# Autodesk Inventor assembly: Assembly
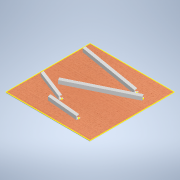
[picture p0: Inventor's stored thumbnail of the model, 180x180]
Saved by Autodesk Inventor 2020 (Build 240168000, 168)
## iProperties
Created: 2020-02-20
Part Number: Assembly
Document SubType Name: Assembly
Designer: brand
Author: brand
## Documents named in this file (3)
- C:\Users\brand\Documents\Longhorn 3D Printing\Week1\Inventor\Assembly.iam
- C:\Users\brand\Documents\Longhorn 3D Printing\Week1\Inventor\Base.ipt
- C:\Users\brand\Documents\Longhorn 3D Printing\Week1\Inventor\StraightTrackv2.ipt
## Components (7 placed, 2 different names)
1. Base:1 — Mate:1, Mate:2, Mate:3, Mate:4, Mate:5, Mate:6
2. StraightTrackv2:1 — Mate:1, Rigid:1
3. StraightTrackv2:2 — Mate:2, Rigid:1
4. StraightTrackv2:3 — Mate:5
5. StraightTrackv2:4 — Mate:3, Mate:7, Flush:1
6. StraightTrackv2:5 — Mate:6, Mate:7, Flush:1
7. StraightTrackv2:6 — Mate:4
## Relationships (9: Mate 7, WeldJoint 1, Flush 1)
- Mate:1: Base:1 ↔ StraightTrackv2:1
- Mate:2: Base:1 ↔ StraightTrackv2:2
- Rigid:1 [WeldJoint]: StraightTrackv2:1 ↔ StraightTrackv2:2
- Mate:3: Base:1 ↔ StraightTrackv2:4
- Mate:4: Base:1 ↔ StraightTrackv2:6
- Mate:5: Base:1 ↔ StraightTrackv2:3
- Mate:6: Base:1 ↔ StraightTrackv2:5
- Mate:7: StraightTrackv2:4 ↔ StraightTrackv2:5
- Flush:1: StraightTrackv2:4 ↔ StraightTrackv2:5
